# Autodesk Inventor assembly: rocker_right
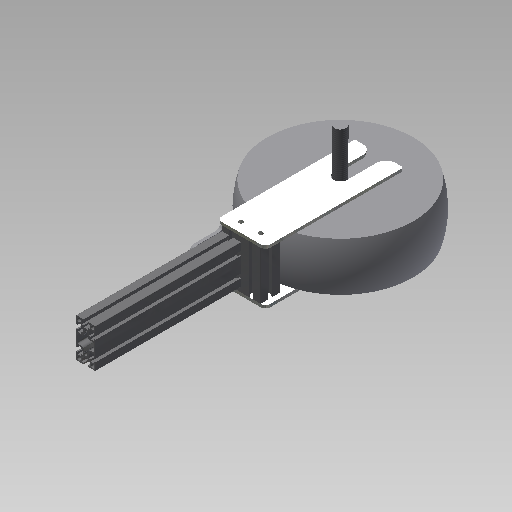
[picture p0: Inventor's stored thumbnail of the model, 512x512]
Saved by Autodesk Inventor 2021.2 (Build 252289000, 289)
## iProperties
Created: 2021-05-27
Part Number: rocker_right
Document SubType Name: Assembly
Designer: gisen
Author: gisen
## Documents named in this file (4)
- C:\Users\gisen\workspace\beetle_inventor_model\suspension\rocker_right.iam
- C:\Users\gisen\workspace\beetle_inventor_model\suspension\wheel_with_mounts_right.iam
- C:\Users\gisen\workspace\beetle_inventor_model\suspension\AFS-2040-4-150_right.ipt
- C:\Users\gisen\workspace\beetle_inventor_model\suspension\wheel_frame_mount_right.ipt
## Components (3 placed, 2 different names)
1. wheel_with_mounts_right:1 [sub-assembly] — メイト:2, メイト:1, フラッシュ:1, メイト:5
2. Part1:1 — メイト:2, メイト:1, フラッシュ:1, メイト:6, メイト:4, メイト:3
3. Part1:2 — メイト:6, メイト:5, メイト:4, メイト:3
## Relationships (7: Mate 6, Flush 1)
- メイト:2 [Mate]: wheel_with_mounts_right:1 ↔ Part1:1
- メイト:1 [Mate]: wheel_with_mounts_right:1 ↔ Part1:1
- フラッシュ:1 [Flush]: wheel_with_mounts_right:1 ↔ Part1:1
- メイト:6 [Mate] (-10 mm): Part1:1 ↔ Part1:2
- メイト:5 [Mate] (-10 mm): wheel_with_mounts_right:1 ↔ Part1:2
- メイト:4 [Mate] (-10 mm): Part1:1 ↔ Part1:2
- メイト:3 [Mate]: Part1:1 ↔ Part1:2
